# Autodesk Inventor assembly: ElectricHousing
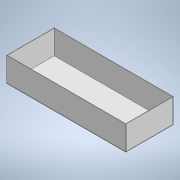
[picture p0: Inventor's stored thumbnail of the model, 180x180]
Saved by Autodesk Inventor 2020 (Build 240168000, 168)
## iProperties
Created: 2021-11-12
Part Number: ElectricHousing
Document SubType Name: Assembly
Designer: 17185
Author: 17185
## Documents named in this file (4)
- C:\Users\17185\Desktop\chassis draft\ElectronicsHousing\ElectronicsCasing.iam
- C:\Users\17185\Desktop\chassis draft\ElectronicsHousing\2.5ftX6in.ipt
- C:\Users\17185\Desktop\chassis draft\ElectronicsHousing\2.5ftX12in.ipt
- C:\Users\17185\Desktop\chassis draft\ElectronicsHousing\12inX6in.ipt
## Components (5 placed, 3 different names)
1. 2.5ftX12in:1 — Flush:10, Flush:11, Mate:5, Flush:12, Mate:6, Flush:13, Flush:15, Mate:8
2. 2.5ftX6in:1 — Flush:10, Flush:11, Mate:5, Mate:7, Mate:9
3. 2.5ftX6in:2 — Flush:12, Mate:6, Flush:14
4. 12inX6in:1 — Flush:13, Mate:7, Flush:14
5. 12inX6in:2 — Flush:15, Mate:8, Mate:9
## Relationships (11: Flush 6, Mate 5)
- Flush:10: 2.5ftX12in:1 ↔ 2.5ftX6in:1
- Flush:11: 2.5ftX12in:1 ↔ 2.5ftX6in:1
- Mate:5: 2.5ftX12in:1 ↔ 2.5ftX6in:1
- Flush:12: 2.5ftX12in:1 ↔ 2.5ftX6in:2
- Mate:6: 2.5ftX12in:1 ↔ 2.5ftX6in:2
- Flush:13: 2.5ftX12in:1 ↔ 12inX6in:1
- Mate:7: 2.5ftX6in:1 ↔ 12inX6in:1
- Flush:14: 2.5ftX6in:2 ↔ 12inX6in:1
- Flush:15: 2.5ftX12in:1 ↔ 12inX6in:2
- Mate:8: 2.5ftX12in:1 ↔ 12inX6in:2
- Mate:9: 2.5ftX6in:1 ↔ 12inX6in:2
